# Autodesk Inventor assembly: ASY GnG station
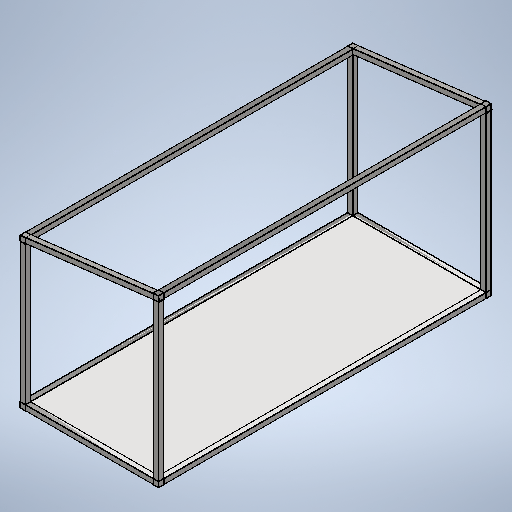
[picture p0: Inventor's stored thumbnail of the model, 512x512]
Saved by Autodesk Inventor 2025 (Build 290162010, 162A)
## iProperties
Created: 2025-09-20
Part Number: ASY GnG station
Document SubType Name: Assembly
Designer: admin
Mass: 766899 g
Surface Area: 646346 cm^2
Volume: 96834.3 cm^3
Density: 7.91971 g/cm^3
Author: admin
## Documents named in this file (3)
- C:\Users\admin\Yandex.Disk\home pc\Inventor\GnG_Gantul_hill\ASY GnG station.iam
- C:\Users\admin\Yandex.Disk\home pc\Inventor\GnG_Gantul_hill\AST GnG frame.iam
- C:\Users\admin\Yandex.Disk\home pc\Inventor\GnG_Gantul_hill\GnG floor sheet 1.ipt
## Components (2 placed, 2 different names)
1. AST GnG frame:1 [sub-assembly] — Flush:1, Flush:2, Flush:3
2. Part1:1 — Flush:1, Flush:2, Flush:3
## Relationships (3: Flush 3)
- Flush:1: AST GnG frame:1 ↔ Part1:1
- Flush:2: AST GnG frame:1 ↔ Part1:1
- Flush:3: AST GnG frame:1 ↔ Part1:1
